# Autodesk Inventor assembly: Pick_&_Place_Nozzle_Assembly
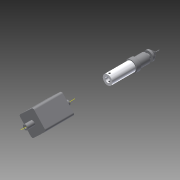
[picture p0: Inventor's stored thumbnail of the model, 180x180]
Saved by Autodesk Inventor 2015 (Build 190159000, 159)
## iProperties
Created: 2015-01-06
Part Number: Pick_&_Place_Nozzle_Assembly
Document SubType Name: Assembly
Designer: ice
Author: ice
## Documents named in this file (6)
- C:\Users\ice\Desktop\PICK\Inventor\Pick_&_Place_Nozzle_Assembly.iam
- C:\Users\ice\Desktop\PICK\Inventor\Extender.ipt
- C:\Users\ice\Desktop\PICK\Inventor\Magnet.ipt
- C:\Users\ice\Desktop\PICK\Inventor\Rubber_Sea_2.5X1N70l##.ipt
- C:\Users\ice\Desktop\PICK\Inventor\Nozzle.ipt
- C:\Users\ice\Desktop\PICK\Inventor\NEMA8.ipt
## Components (6 placed, 5 different names)
1. Extender:1 — Mate:2, Mate:3, Mate:4, Mate:5
2. Magnet:1
3. Rubber_Sea_2.5X1N70l##:1 — Mate:2
4. Rubber_Sea_2.5X1N70l##:2 — Mate:3
5. Nozzle:1 — Mate:4
6. NEMA8:1 — Mate:5
## Relationships (6: Mate 5, Flush 1)
- [Mate]: Extender:1 ↔ Magnet:1
- [Flush]: Extender:1 ↔ Magnet:1
- Mate:2: Extender:1 ↔ Rubber_Sea_2.5X1N70l##:1
- Mate:3: Extender:1 ↔ Rubber_Sea_2.5X1N70l##:2
- Mate:4: Extender:1 ↔ Nozzle:1
- Mate:5: Extender:1 ↔ NEMA8:1
